# Autodesk Inventor assembly: artifact-v2
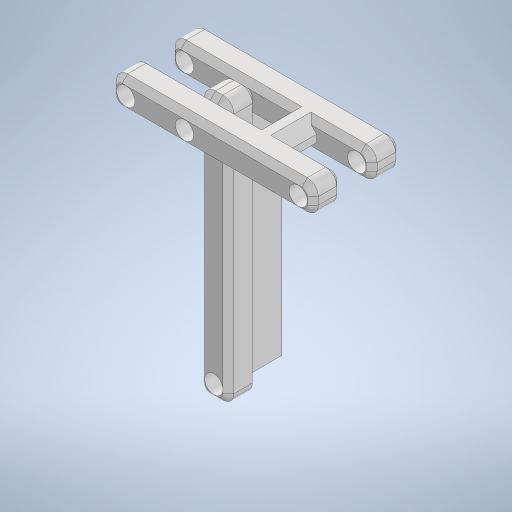
[picture p0: Inventor's stored thumbnail of the model, 512x512]
Saved by Autodesk Inventor 2024.1 (Build 281209000, 209)
## iProperties
Created: 2025-07-06
Part Number: artifact-v2
Document SubType Name: Assembly
Designer: iwheard
Author: iwheard
## Documents named in this file (3)
- C:\Users\iwheard\Documents\0004-CAD\3D-cad-main\the-artifact\artifact-v2.iam
- C:\Users\iwheard\Documents\0004-CAD\3D-cad-main\the-artifact\base.ipt
- C:\Users\iwheard\Documents\0004-CAD\3D-cad-main\the-artifact\cross-beam.ipt
## Components (2 placed, 2 different names)
1. base:1 — Flush:1
2. cross-beam:1 — Flush:1
## Relationships (1: Flush 1)
- Flush:1: base:1 ↔ cross-beam:1
